# Autodesk Inventor assembly: POM_T5_10
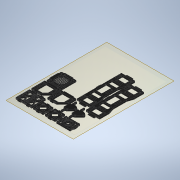
[picture p0: Inventor's stored thumbnail of the model, 180x180]
Saved by Autodesk Inventor 2020 (Build 240168000, 168)
## iProperties
Created: 2021-08-27
Part Number: POM_T5_10
Document SubType Name: Assembly
Designer: Masato
Author: Masato
## Documents named in this file (9)
- C:\Users\naoki\Documents\Inventor\CitBrains\git_clone\OpenPlatform4_1\A_T5_POM\OpenPlatform_ver3_0\cam\POM_T5_10.iam
- C:\Users\naoki\Documents\Inventor\CitBrains\git_clone\OpenPlatform4_1\A_T5_POM\OpenPlatform_ver3_0\cam\Disposable_Board.ipt
- C:\Users\naoki\Documents\Inventor\CitBrains\git_clone\OpenPlatform4_1\A_T5_POM\OpenPlatform_ver3_0\UpperBody\Arm\ForeArm_diagonal.ipt
- C:\Users\naoki\Documents\Inventor\CitBrains\git_clone\OpenPlatform4_1\A_T5_POM\OpenPlatform_ver3_0\UpperBody\Arm\UpperArm_diagonal.ipt
- C:\Users\naoki\Documents\Inventor\CitBrains\git_clone\OpenPlatform4_1\A_T5_POM\OpenPlatform_ver3_0\UpperBody\Head\Head_horn_frame.ipt
- C:\Users\naoki\Documents\Inventor\CitBrains\git_clone\OpenPlatform4_1\A_T5_POM\OpenPlatform_ver3_0\UpperBody\Head\Head_diagonal.ipt
- C:\Users\naoki\Documents\Inventor\CitBrains\git_clone\OpenPlatform4_1\A_T5_POM\OpenPlatform_ver3_0\UpperBody\Head\Camera_root_frame.ipt
- C:\Users\naoki\Documents\Inventor\CitBrains\git_clone\OpenPlatform4_1\A_T5_POM\OpenPlatform_ver3_0\UpperBody\Head\Camera_side_frame.ipt
- C:\Users\naoki\Documents\Inventor\CitBrains\git_clone\OpenPlatform4_1\A_T5_POM\OpenPlatform_ver3_0\UpperBody\Trunk\Trunk_chest_frame.ipt
## Components (13 placed, 8 different names)
1. Disposable_Board:1 — メイト:2, メイト:1, フラッシュ:1, フラッシュ:2, メイト:4, メイト:5, メイト:6, メイト:7, メイト:8, メイト:9, メイト:10, フラッシュ:3, フラッシュ:4, フラッシュ:5, フラッシュ:6, フラッシュ:7, フラッシュ:8, フラッシュ:9, メイト:17, メイト:18, メイト:19, メイト:24, メイト:25, メイト:26, フラッシュ:11
2. ForeArm_diagonal:1 — メイト:8, フラッシュ:9, メイト:15, メイト:16, フラッシュ:10, メイト:23
3. ForeArm_diagonal:2 — メイト:9, メイト:16, フラッシュ:10, メイト:20, メイト:28
4. UpperArm_diagonal:1 — メイト:7, フラッシュ:7, メイト:13, メイト:14, メイト:21
5. UpperArm_diagonal:2 — メイト:6, フラッシュ:6, メイト:12, メイト:13
6. Head_horn_frame:1 — メイト:10, フラッシュ:8, メイト:14, メイト:22
7. Head_diagonal:1 — メイト:4, フラッシュ:3, フラッシュ:4, メイト:11, メイト:15
8. Head_diagonal:2 — メイト:5, フラッシュ:5, メイト:11, メイト:12
9. Camera_root_frame:1 — メイト:19, メイト:23, メイト:24
10. Camera_side_frame:1 — メイト:18, メイト:22, 正接:1, 正接:2
11. Camera_side_frame:2 — メイト:17, メイト:20, メイト:21, 正接:1
12. Trunk_chest_frame:1 — メイト:25, フラッシュ:11, 正接:2, メイト:27
13. Trunk_chest_frame:2 — メイト:26, メイト:27, メイト:28
## Relationships (40: Mate 27, Flush 11, Tangent 2)
- メイト:2 [Mate]: Disposable_Board:1
- メイト:1 [Mate]: Disposable_Board:1
- フラッシュ:1 [Flush]: Disposable_Board:1
- フラッシュ:2 [Flush]: Disposable_Board:1
- メイト:4 [Mate]: Disposable_Board:1 ↔ Head_diagonal:1
- メイト:5 [Mate]: Disposable_Board:1 ↔ Head_diagonal:2
- メイト:6 [Mate]: Disposable_Board:1 ↔ UpperArm_diagonal:2
- メイト:7 [Mate]: Disposable_Board:1 ↔ UpperArm_diagonal:1
- メイト:8 [Mate]: Disposable_Board:1 ↔ ForeArm_diagonal:1
- メイト:9 [Mate]: Disposable_Board:1 ↔ ForeArm_diagonal:2
- メイト:10 [Mate]: Disposable_Board:1 ↔ Head_horn_frame:1
- フラッシュ:3 [Flush] (2.5 mm): Disposable_Board:1 ↔ Head_diagonal:1
- フラッシュ:4 [Flush] (2.5 mm): Disposable_Board:1 ↔ Head_diagonal:1
- フラッシュ:5 [Flush] (2.5 mm): Disposable_Board:1 ↔ Head_diagonal:2
- メイト:11 [Mate] (2.5 mm): Head_diagonal:1 ↔ Head_diagonal:2
- フラッシュ:6 [Flush] (2.5 mm): Disposable_Board:1 ↔ UpperArm_diagonal:2
- メイト:12 [Mate] (2.5 mm): UpperArm_diagonal:2 ↔ Head_diagonal:2
- フラッシュ:7 [Flush] (2.5 mm): Disposable_Board:1 ↔ UpperArm_diagonal:1
- メイト:13 [Mate] (2.5 mm): UpperArm_diagonal:1 ↔ UpperArm_diagonal:2
- フラッシュ:8 [Flush] (2.5 mm): Disposable_Board:1 ↔ Head_horn_frame:1
- メイト:14 [Mate] (2.5 mm): UpperArm_diagonal:1 ↔ Head_horn_frame:1
- フラッシュ:9 [Flush] (2.5 mm): Disposable_Board:1 ↔ ForeArm_diagonal:1
- メイト:15 [Mate] (2.5 mm): ForeArm_diagonal:1 ↔ Head_diagonal:1
- メイト:16 [Mate] (2.5 mm): ForeArm_diagonal:1 ↔ ForeArm_diagonal:2
- フラッシュ:10 [Flush]: ForeArm_diagonal:1 ↔ ForeArm_diagonal:2
- メイト:17 [Mate]: Disposable_Board:1 ↔ Camera_side_frame:2
- メイト:18 [Mate]: Disposable_Board:1 ↔ Camera_side_frame:1
- メイト:19 [Mate]: Disposable_Board:1 ↔ Camera_root_frame:1
- メイト:20 [Mate] (2.5 mm): ForeArm_diagonal:2 ↔ Camera_side_frame:2
- メイト:21 [Mate] (2.5 mm): UpperArm_diagonal:1 ↔ Camera_side_frame:2
- メイト:22 [Mate] (2.5 mm): Head_horn_frame:1 ↔ Camera_side_frame:1
- 正接:1 [Tangent] (2.5 mm): Camera_side_frame:1 ↔ Camera_side_frame:2
- メイト:23 [Mate] (2.5 mm): ForeArm_diagonal:1 ↔ Camera_root_frame:1
- メイト:24 [Mate] (2.5 mm): Disposable_Board:1 ↔ Camera_root_frame:1
- メイト:25 [Mate]: Disposable_Board:1 ↔ Trunk_chest_frame:1
- メイト:26 [Mate]: Disposable_Board:1 ↔ Trunk_chest_frame:2
- フラッシュ:11 [Flush] (3 mm): Disposable_Board:1 ↔ Trunk_chest_frame:1
- 正接:2 [Tangent] (3 mm): Camera_side_frame:1 ↔ Trunk_chest_frame:1
- メイト:27 [Mate] (2.5 mm): Trunk_chest_frame:1 ↔ Trunk_chest_frame:2
- メイト:28 [Mate] (2 mm): ForeArm_diagonal:2 ↔ Trunk_chest_frame:2
